# Autodesk Inventor assembly: Assembly2
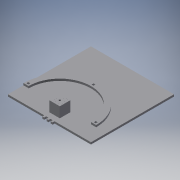
[picture p0: Inventor's stored thumbnail of the model, 180x180]
Saved by Autodesk Inventor 2018 (Build 220112000, 112)
## iProperties
Created: 2018-04-30
Part Number: Assembly2
Document SubType Name: Assembly
Designer: Administrator
Author: Administrator
## Documents named in this file (6)
- C:\Users\jerrywang\Documents\Assembly2.iam
- C:\Users\jerrywang\Documents\Part7.ipt
- C:\Users\jerrywang\Documents\Part8.ipt
- C:\Users\jerrywang\Documents\Part9.ipt
- C:\Users\jerrywang\Documents\Part10.ipt
- C:\Users\jerrywang\Documents\Part11.ipt
## Components (7 placed, 5 different names)
1. Part7:1 — Flush:10, Mate:1, Flush:17, Mate:3
2. Part8:2 — Flush:1, Flush:4, Flush:7, Mate:1, Flush:18, Flush:19, Mate:3
3. Part8:3 — Flush:1, Flush:3, Flush:4, Flush:7, Flush:12, Flush:13, Flush:15
4. Part8:4 — Flush:3, Flush:10, Flush:11, Flush:14, Flush:18, Flush:19, Flush:20
5. Part9:1 — Flush:11, Flush:12, Flush:13, Flush:16, Mate:2
6. Part10:1 — Flush:14, Flush:15, Flush:16
7. Part11:1 — Flush:17, Mate:2, Flush:20
## Relationships (18: Flush 15, Mate 3)
- Flush:1: Part8:2 ↔ Part8:3
- Flush:3: Part8:3 ↔ Part8:4
- Flush:4: Part8:2 ↔ Part8:3
- Flush:7: Part8:2 ↔ Part8:3
- Flush:10: Part7:1 ↔ Part8:4
- Mate:1: Part7:1 ↔ Part8:2
- Flush:11: Part8:4 ↔ Part9:1
- Flush:12: Part8:3 ↔ Part9:1
- Flush:13: Part8:3 ↔ Part9:1
- Flush:14: Part8:4 ↔ Part10:1
- Flush:15: Part8:3 ↔ Part10:1
- Flush:16: Part9:1 ↔ Part10:1
- Flush:17 (12.7 mm): Part7:1 ↔ Part11:1
- Mate:2 (63.5 mm): Part9:1 ↔ Part11:1
- Flush:18: Part8:2 ↔ Part8:4
- Flush:19: Part8:2 ↔ Part8:4
- Mate:3: Part7:1 ↔ Part8:2
- Flush:20 (12.7 mm): Part8:4 ↔ Part11:1
